# Autodesk Inventor assembly: upper_leg
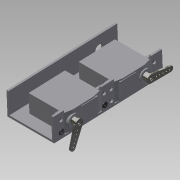
[picture p0: Inventor's stored thumbnail of the model, 180x180]
Saved by Autodesk Inventor 2015 (Build 190159000, 159)
## iProperties
Created: 2014-06-08
Part Number: upper_leg
Document SubType Name: Assembly
Designer: L
Author: L
## Documents named in this file (3)
- D:\Documents\GitHub\SolidModels\stag_v2_01_pre_alpha\upper_leg.iam
- D:\Documents\GitHub\SolidModels\stag_v2_01_pre_alpha\upper_leg.ipt
- D:\Documents\GitHub\SolidModels\stag_v2_01_pre_alpha\ServoAssembly.iam
## Components (3 placed, 2 different names)
1. upper_leg:1 — Mate:1, Mate:2, Mate:3, Mate:4, Mate:5, Mate:6
2. ServoAssembly:1 [sub-assembly] — Mate:1, Mate:2, Mate:3
3. ServoAssembly:2 [sub-assembly] — Mate:4, Mate:5, Mate:6
## Relationships (6: Mate 6)
- Mate:1: upper_leg:1 ↔ ServoAssembly:1
- Mate:2: upper_leg:1 ↔ ServoAssembly:1
- Mate:3: upper_leg:1 ↔ ServoAssembly:1
- Mate:4: upper_leg:1 ↔ ServoAssembly:2
- Mate:5: upper_leg:1 ↔ ServoAssembly:2
- Mate:6: upper_leg:1 ↔ ServoAssembly:2
